# Autodesk Inventor assembly: interface
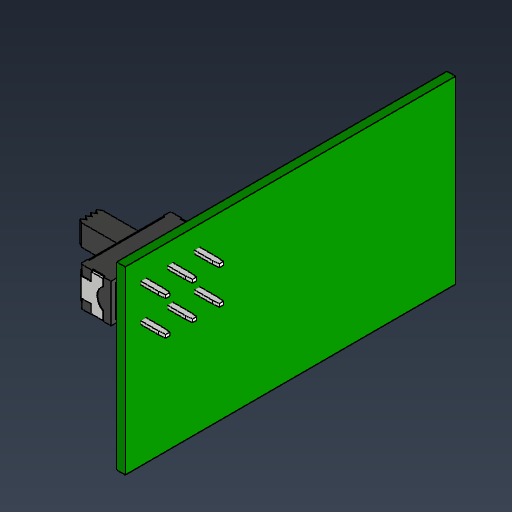
[picture p0: Inventor's stored thumbnail of the model, 512x512]
Saved by Autodesk Inventor 2026.2 (Build 302298010, 298A)
## iProperties
Created: 2026-03-25
Part Number: interface
Document SubType Name: Assembly
Designer: szymo
Author: szymo
## Documents named in this file (3)
- D:\tech\robotyka\robots\evangelion-turbo\inventor-project\interface.iam
- D:\tech\robotyka\robots\evangelion-turbo\inventor-project\microswitch_EG1271A\microswitch_EG1271A\microswitch_EG1271A.ipt
- D:\tech\robotyka\robots\evangelion-turbo\inventor-project\interface-pcb.ipt
## Components (2 placed, 2 different names)
1. interface-pcb:1 — Mate:1, Mate:2, Flush:2, Mate:3
2. microswitch_EG1271A:1
## Relationships (4: Mate 3, Flush 1)
- Mate:1: interface-pcb:1
- Mate:2: interface-pcb:1
- Flush:2: interface-pcb:1
- Mate:3: interface-pcb:1
